# Autodesk Inventor assembly: Female_Tail_Assembly
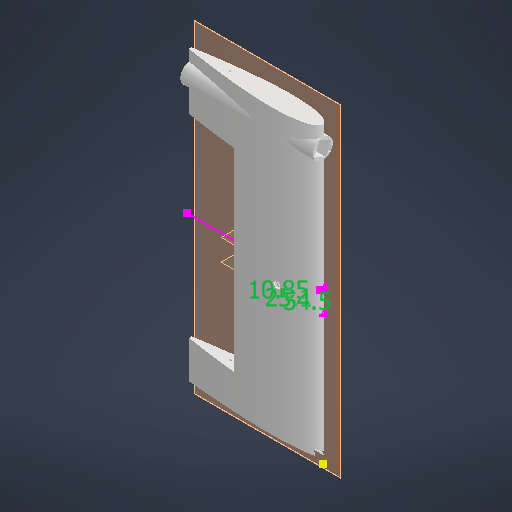
[picture p0: Inventor's stored thumbnail of the model, 512x512]
Saved by Autodesk Inventor 2026 (Build 300175050, 175E)
## iProperties
Created: 2026-07-06
Part Number: Female_Tail_Assembly
Document SubType Name: Assembly
Designer: Delbe
Author: Delbe
## Documents named in this file (3)
- C:\GitHub\SWIFT-UAV\System_development\Pelican\structural_model\v0.3.0\Parts\Delb_Parts\Female_Tail_Assembly.iam
- C:\GitHub\SWIFT-UAV\System_development\Pelican\structural_model\v0.3.0\Parts\Delb_Parts\Female_Tail_Female_Connector.ipt
- C:\GitHub\SWIFT-UAV\System_development\Pelican\structural_model\v0.3.0\Parts\Delb_Parts\Female_Tail_Male_Connector.ipt
## Components (2 placed, 2 different names)
1. Female_Tail_Female_Connector:1 — Mate:1
2. Female_Tail_Male_Connector:1 — Mate:1
## Relationships (1: Mate 1)
- Mate:1: Female_Tail_Female_Connector:1 ↔ Female_Tail_Male_Connector:1
